# Autodesk Inventor assembly: Overlay of Wheel Basses
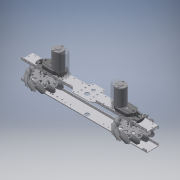
[picture p0: Inventor's stored thumbnail of the model, 180x180]
Saved by Autodesk Inventor 2018 (Build 220112000, 112)
## iProperties
Created: 2018-01-16
Part Number: Overlay of Wheel Basses
Document SubType Name: Assembly
Designer: Apple
Author: Apple
## Documents named in this file (3)
- C:\Users\Apple\Documents\Inventor\2018 PowerUp\Overlay of Wheel Basses.iam
- C:\Users\Apple\Documents\Inventor\2018 PowerUp\2017 Plate with 2018 boxes.iam
- C:\Users\Apple\Documents\Inventor\2018 PowerUp\2016 plate with 2018 boxes.iam
## Components (2 placed, 2 different names)
1. 2017 Plate with 2018 boxes:1 [sub-assembly] — Flush:1, Flush:2, Flush:3
2. 2016 plate with 2018 boxes:1 [sub-assembly] — Flush:1, Flush:2, Flush:3
## Relationships (3: Flush 3)
- Flush:1: 2017 Plate with 2018 boxes:1 ↔ 2016 plate with 2018 boxes:1
- Flush:2: 2017 Plate with 2018 boxes:1 ↔ 2016 plate with 2018 boxes:1
- Flush:3: 2017 Plate with 2018 boxes:1 ↔ 2016 plate with 2018 boxes:1
